# Autodesk Inventor assembly: Assembly1
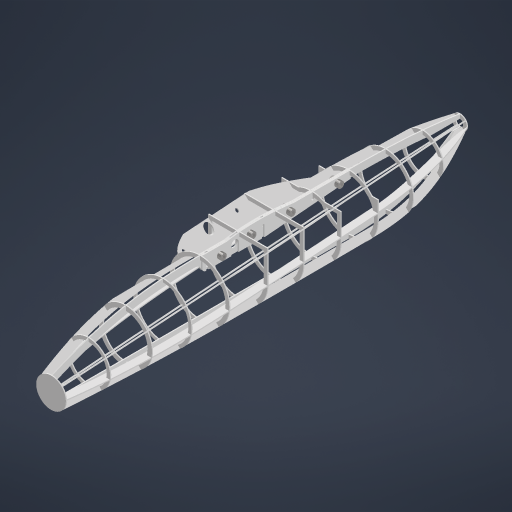
[picture p0: Inventor's stored thumbnail of the model, 512x512]
Saved by Autodesk Inventor 2023.2 (Build 272271000, 271)
## iProperties
Created: 2023-01-02
Part Number: Assembly1
Document SubType Name: Assembly
Designer: Maciej
Author: Maciej
## Documents named in this file (25)
- C:\Users\Maciej\Desktop\samolot\Solaris\main\new model\Assembly1.iam
- C:\Users\Maciej\Desktop\samolot\Solaris\main\new model\Part1.ipt
- C:\Users\Maciej\Desktop\samolot\Solaris\main\new model\Part2.ipt
- C:\Users\Maciej\Desktop\samolot\Solaris\main\new model\Part3.ipt
- C:\Users\Maciej\Desktop\samolot\Solaris\main\new model\Part4.ipt
- C:\Users\Maciej\Desktop\samolot\Solaris\main\new model\Part5.ipt
- C:\Users\Maciej\Desktop\samolot\Solaris\main\new model\Part6.ipt
- C:\Users\Maciej\Desktop\samolot\Solaris\main\new model\Part7.ipt
- C:\Users\Maciej\Desktop\samolot\Solaris\main\new model\Part8.ipt
- C:\Users\Maciej\Desktop\samolot\Solaris\main\new model\Part9.ipt
- C:\Users\Maciej\Desktop\samolot\Solaris\main\new model\Part10.ipt
- C:\Users\Maciej\Desktop\samolot\Solaris\main\new model\Part11.ipt
- C:\Users\Maciej\Desktop\samolot\Solaris\main\new model\Part12.ipt
- C:\Users\Maciej\Desktop\samolot\Solaris\main\new model\Part13.ipt
- C:\Users\Maciej\Desktop\samolot\Solaris\main\new model\Part14.ipt
- C:\Users\Maciej\Desktop\samolot\Solaris\main\new model\Part15.ipt
- C:\Users\Maciej\Desktop\samolot\Solaris\main\new model\Part16.ipt
- C:\Users\Maciej\Desktop\samolot\Solaris\main\new model\Part17.ipt
- C:\Users\Maciej\Desktop\samolot\Solaris\main\new model\Part18.ipt
- C:\Users\Maciej\Desktop\samolot\Solaris\main\new model\Part19.ipt
- C:\Users\Maciej\Desktop\samolot\Solaris\main\new model\Part20.ipt
- C:\Users\Maciej\Desktop\samolot\Solaris\main\new model\Part21.ipt
- C:\Users\Maciej\Desktop\samolot\Solaris\main\new model\Part22.ipt
- C:\Users\Maciej\Documents\Inventor\Content Center Files\R2023\en-US\DIN 912\DIN 912 - M5 x 0,8 x 8 x 6.ipt
- C:\Users\Maciej\Documents\Inventor\Content Center Files\R2023\en-US\DIN 934\DIN 934 - M5 x 0,8.ipt
## Components (31 placed, 24 different names)
1. Part1:1
2. Part2:1
3. Part3:1
4. Part4:1
5. Part5:1
6. Part6:1
7. Part7:1
8. Part8:1
9. Part9:1
10. Part10:1
11. Part11:1
12. Part12:1
13. Part13:1
14. Part14:1
15. Part15:1
16. Part16:1
17. Part17:1
18. Part18:1
19. Part19:1
20. Part20:1
21. Part21:1 — Insert:1, Insert:2, Insert:3, Insert:4
22. Part22:1 — Mate:4, Mate:6, Mate:8, Mate:10
23. DIN 912 - replaced by DIN EN ISO 4762 M5 x 8:1 — Insert:1, Mate:7
24. DIN 912 - replaced by DIN EN ISO 4762 M5 x 8:2 — Insert:2, Mate:9
25. DIN 912 - replaced by DIN EN ISO 4762 M5 x 8:3 — Insert:3, Mate:3
26. DIN 912 - replaced by DIN EN ISO 4762 M5 x 8:4 — Insert:4, Mate:1, Mate:2, Mate:5
27. DIN 934 - replaced by DIN EN 24032/28673/28674 M5:1 — Mate:1, Mate:2
28. DIN 934 - replaced by DIN EN 24032/28673/28674 M5:2 — Mate:3, Mate:4
29. DIN 934 - replaced by DIN EN 24032/28673/28674 M5:3 — Mate:5, Mate:6
30. DIN 934 - replaced by DIN EN 24032/28673/28674 M5:4 — Mate:7, Mate:8
31. DIN 934 - replaced by DIN EN 24032/28673/28674 M5:5 — Mate:9, Mate:10
## Relationships (14: Mate 10, Insert 4)
- Insert:1: Part21:1 ↔ DIN 912 - replaced by DIN EN ISO 4762 M5 x 8:1
- Insert:2: Part21:1 ↔ DIN 912 - replaced by DIN EN ISO 4762 M5 x 8:2
- Insert:3: Part21:1 ↔ DIN 912 - replaced by DIN EN ISO 4762 M5 x 8:3
- Insert:4: Part21:1 ↔ DIN 912 - replaced by DIN EN ISO 4762 M5 x 8:4
- Mate:1: DIN 912 - replaced by DIN EN ISO 4762 M5 x 8:4 ↔ DIN 934 - replaced by DIN EN 24032/28673/28674 M5:1
- Mate:2: DIN 912 - replaced by DIN EN ISO 4762 M5 x 8:4 ↔ DIN 934 - replaced by DIN EN 24032/28673/28674 M5:1
- Mate:3: DIN 912 - replaced by DIN EN ISO 4762 M5 x 8:3 ↔ DIN 934 - replaced by DIN EN 24032/28673/28674 M5:2
- Mate:4: Part22:1 ↔ DIN 934 - replaced by DIN EN 24032/28673/28674 M5:2
- Mate:5: DIN 912 - replaced by DIN EN ISO 4762 M5 x 8:4 ↔ DIN 934 - replaced by DIN EN 24032/28673/28674 M5:3
- Mate:6: Part22:1 ↔ DIN 934 - replaced by DIN EN 24032/28673/28674 M5:3
- Mate:7: DIN 912 - replaced by DIN EN ISO 4762 M5 x 8:1 ↔ DIN 934 - replaced by DIN EN 24032/28673/28674 M5:4
- Mate:8: Part22:1 ↔ DIN 934 - replaced by DIN EN 24032/28673/28674 M5:4
- Mate:9: DIN 912 - replaced by DIN EN ISO 4762 M5 x 8:2 ↔ DIN 934 - replaced by DIN EN 24032/28673/28674 M5:5
- Mate:10: Part22:1 ↔ DIN 934 - replaced by DIN EN 24032/28673/28674 M5:5
